# Autodesk Inventor assembly: Ensemble
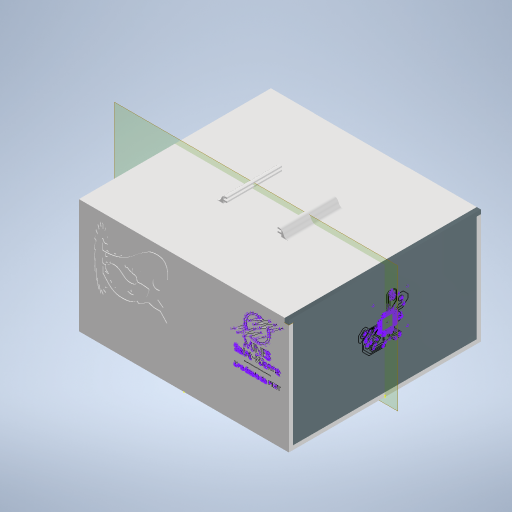
[picture p0: Inventor's stored thumbnail of the model, 512x512]
Saved by Autodesk Inventor 2023 (Build 270158000, 158)
## iProperties
Created: 2023-03-24
Part Number: Ensemble
Document SubType Name: Assembly
Designer: eleves
Author: eleves
## Documents named in this file (4)
- C:\Users\eleves\Desktop\PE-SM\3D\Ensemble.iam
- C:\Users\eleves\Desktop\PE-SM\3D\PE.ipt
- C:\Users\eleves\Desktop\PE-SM\3D\Nucleo\NUCLEO-F429ZI--3DModel-STEP-56544.ipt
- C:\Users\eleves\Desktop\PE-SM\3D\Door.ipt
## Components (3 placed, 3 different names)
1. PE:1 — Placage:1, Placage:2, Placage:3, Affleurement:1, Affleurement:2
2. NUCLEO-F429ZI--3DModel-STEP-56544:1 — Placage:1, Placage:2, Placage:3
3. Door:1 — Affleurement:1, Affleurement:2
## Relationships (5: Mate 3, Flush 2)
- Placage:1 [Mate] (15 mm): PE:1 ↔ NUCLEO-F429ZI--3DModel-STEP-56544:1
- Placage:2 [Mate]: PE:1 ↔ NUCLEO-F429ZI--3DModel-STEP-56544:1
- Placage:3 [Mate]: PE:1 ↔ NUCLEO-F429ZI--3DModel-STEP-56544:1
- Affleurement:1 [Flush]: PE:1 ↔ Door:1
- Affleurement:2 [Flush]: PE:1 ↔ Door:1
